# Autodesk Inventor assembly: Flexiwheel
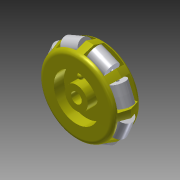
[picture p0: Inventor's stored thumbnail of the model, 180x180]
Saved by Autodesk Inventor 2014 (Build 180170000, 170)
## iProperties
Created: 2014-02-14
Part Number: Flexiwheel
Document SubType Name: Assembly
Designer: Spooner
Author: Spooner
## Documents named in this file (3)
- C:\Users\Spooner\Documents\Inventor\FerretBall Robot\3Pod\Inventor 2014 Files\Flexiwheel.iam
- C:\Users\Spooner\Documents\Inventor\FerretBall Robot\3Pod\Inventor 2014 Files\Flexiwheel - Half Wheel.ipt
- C:\Users\Spooner\Documents\Inventor\FerretBall Robot\3Pod\Inventor 2014 Files\Flexiwheel Roller.ipt
## Components (10 placed, 2 different names)
1. Flexiwheel - Half Wheel:1 — Insert:9, Angle:1
2. Flexiwheel - Half Wheel:2 — Insert:1, Insert:2, Insert:3, Insert:4, Insert:5, Insert:6, Insert:7, Insert:8, Insert:9, Angle:1
3. Flexiwheel Roller:1 — Insert:4
4. Flexiwheel Roller:2 — Insert:5
5. Flexiwheel Roller:3 — Insert:6
6. Flexiwheel Roller:4 — Insert:8
7. Flexiwheel Roller:5 — Insert:7
8. Flexiwheel Roller:6 — Insert:3
9. Flexiwheel Roller:7 — Insert:2
10. Flexiwheel Roller:8 — Insert:1
## Relationships (10: Insert 9, Angle 1)
- Insert:1: Flexiwheel - Half Wheel:2 ↔ Flexiwheel Roller:8
- Insert:2: Flexiwheel - Half Wheel:2 ↔ Flexiwheel Roller:7
- Insert:3: Flexiwheel - Half Wheel:2 ↔ Flexiwheel Roller:6
- Insert:4: Flexiwheel - Half Wheel:2 ↔ Flexiwheel Roller:1
- Insert:5: Flexiwheel - Half Wheel:2 ↔ Flexiwheel Roller:2
- Insert:6: Flexiwheel - Half Wheel:2 ↔ Flexiwheel Roller:3
- Insert:7: Flexiwheel - Half Wheel:2 ↔ Flexiwheel Roller:5
- Insert:8: Flexiwheel - Half Wheel:2 ↔ Flexiwheel Roller:4
- Insert:9: Flexiwheel - Half Wheel:1 ↔ Flexiwheel - Half Wheel:2
- Angle:1 (0 deg): Flexiwheel - Half Wheel:1 ↔ Flexiwheel - Half Wheel:2
